# Autodesk Inventor assembly: Manipulator
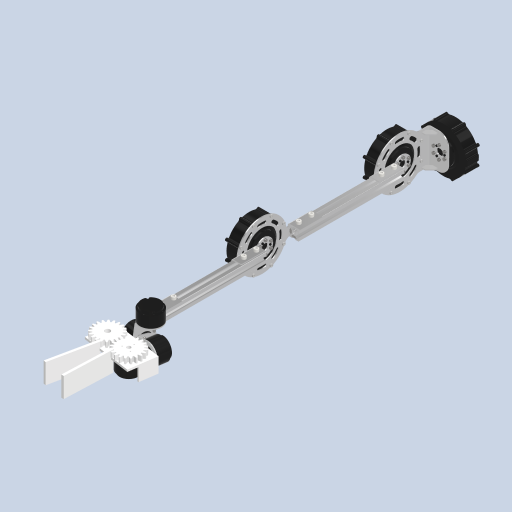
[picture p0: Inventor's stored thumbnail of the model, 512x512]
Saved by Autodesk Inventor 2023 (Build 270158000, 158)
## iProperties
Created: 2024-11-08
Part Number: Manipulator
Document SubType Name: Assembly
Designer: kiyo
Author: kiyo
## Documents named in this file (19)
- D:\GitHub\inventor\syu-si\OfficeRobot\Manipulator\Manipulator.iam
- D:\GitHub\inventor\syu-si\OfficeRobot\ReadyMade\Steadywin\GIM8108-8.iam
- D:\GitHub\inventor\syu-si\OfficeRobot\Manipulator\elbow-pitch-bracket.ipt
- D:\GitHub\inventor\syu-si\OfficeRobot\Manipulator\Hand.iam
- D:\GitHub\inventor\syu-si\OfficeRobot\ReadyMade\Screw\M3_6mm.ipt
- D:\GitHub\inventor\syu-si\OfficeRobot\ReadyMade\Steadywin\GIM3505-8_with-driver.ipt
- D:\GitHub\inventor\syu-si\OfficeRobot\Manipulator\wrist_roll_plate.ipt
- D:\GitHub\inventor\syu-si\OfficeRobot\Manipulator\wrist-pitch-plate.ipt
- D:\GitHub\inventor\syu-si\OfficeRobot\Manipulator\wrist-yaw-plate.ipt
- D:\GitHub\inventor\syu-si\OfficeRobot\ReadyMade\Screw\M2-5_6mm.ipt
- D:\GitHub\inventor\syu-si\OfficeRobot\ReadyMade\Screw\CBSH3-8.ipt
- D:\GitHub\inventor\syu-si\OfficeRobot\ReadyMade\Screw\FWSJJ-D5-V2_6-T4_5.ipt
- D:\GitHub\inventor\syu-si\OfficeRobot\ReadyMade\Screw\M2-5_10mm.ipt
- D:\GitHub\inventor\syu-si\OfficeRobot\ReadyMade\Screw\HNTU5-5.ipt
- D:\GitHub\inventor\syu-si\OfficeRobot\Manipulator\pitch_plate_20mm.ipt
- D:\GitHub\inventor\syu-si\OfficeRobot\ReadyMade\Aluminum-frame\HFS5-2020-210-AV10-BV35-CV175-DV200.ipt
- D:\GitHub\inventor\syu-si\OfficeRobot\Manipulator\sholder_roll_bracket.ipt
- D:\GitHub\inventor\syu-si\OfficeRobot\ReadyMade\Screw\SCB5-22.ipt
- D:\GitHub\inventor\syu-si\OfficeRobot\ReadyMade\Screw\SCB5-8.ipt
## Components (110 placed, 18 different names)
1. wrist_roll_plate:1 — 挿入:220, 挿入:227, 挿入:228, 挿入:229, 挿入:230, 挿入:231, 挿入:283, 挿入:284, 挿入:285
2. wrist-pitch-plate:1 — 挿入:211, 挿入:212, 挿入:213, 挿入:217, 挿入:218, 挿入:219, 挿入:220, 挿入:280, 挿入:281, 挿入:282
3. wrist-yaw-plate:1 — 挿入:203, 挿入:204, 挿入:205, 挿入:206, 挿入:207, 挿入:211, メイト:13, メイト:14, フラッシュ:4
4. pitch_plate_20mm:1 — 肩ピッチ, フラッシュ:1, 挿入:355, 挿入:356, 挿入:357, 挿入:358, 挿入:359, 挿入:360
5. pitch_plate_20mm:2 — 挿入:345, 肘ピッチ, フラッシュ:3
6. elbow-pitch-bracket:1 — 挿入:341, 挿入:342, フラッシュ:2, フラッシュ:7, フラッシュ:8
7. sholder_roll_bracket:1 — 挿入:348, 挿入:349, 挿入:350, 挿入:361, 挿入:362, 挿入:363, 挿入:364, 挿入:365, 挿入:366
8. Hand:1 [sub-assembly] — ハンド, 挿入:301
9. HFS5-2020-210-AV10-BV35-CV175-DV200:1 — フラッシュ:1, フラッシュ:2, メイト:19, メイト:20, 角度:35, 角度:36, メイト:21, メイト:22, フラッシュ:9, 角度:37, メイト:23, メイト:24
10. HFS5-2020-210-AV10-BV35-CV175-DV200:2 — フラッシュ:3, 挿入:351, 挿入:352, 角度:27, 角度:28, 挿入:353, 挿入:354, 角度:29, 角度:30, メイト:9, 角度:31, メイト:10, 角度:32, メイト:11, メイト:12, メイト:13, メイト:14, フラッシュ:4, メイト:15, メイト:16, 角度:33, フラッシュ:5, メイト:17, メイト:18, 角度:34, フラッシュ:6
11. M3_6mm:7 — 挿入:337
12. M3_6mm:8 — 挿入:336
13. M3_6mm:9 — 挿入:334
14. M3_6mm:10 — 挿入:338
15. M3_6mm:11 — 挿入:339
16. M3_6mm:12 — 挿入:335
17. M3_6mm:13
18. M3_6mm:14
19. M3_6mm:15
20. M3_6mm:16
21. M3_6mm:17
22. M3_6mm:18
23. M3_6mm:19 — 挿入:358
24. M3_6mm:20 — 挿入:357
25. M3_6mm:21 — 挿入:355
26. M3_6mm:22 — 挿入:356
27. M3_6mm:23 — 挿入:359
28. M3_6mm:24 — 挿入:360
29. M3_6mm:25 — 挿入:361
30. M3_6mm:26 — 挿入:363
31. M3_6mm:27 — 挿入:362
32. M3_6mm:28 — 挿入:364
33. M3_6mm:29 — 挿入:365
34. M3_6mm:30 — 挿入:366
35. CBSH3-8:1 — 挿入:307
36. CBSH3-8:2 — 挿入:308
37. CBSH3-8:3 — 挿入:302
38. CBSH3-8:4 — 挿入:304
39. CBSH3-8:5 — 挿入:309
40. CBSH3-8:6 — 挿入:303
41. CBSH3-8:7 — 挿入:305
42. CBSH3-8:8 — 挿入:306
43. CBSH3-8:9 — 挿入:332
44. CBSH3-8:10 — 挿入:327
45. CBSH3-8:11 — 挿入:330
46. CBSH3-8:12 — 挿入:328
47. CBSH3-8:13 — 挿入:329
48. CBSH3-8:14 — 挿入:331
49. CBSH3-8:15 — 挿入:326
50. CBSH3-8:16 — 挿入:333
51. M2-5_6mm:1 — 挿入:205
52. M2-5_6mm:2 — 挿入:207
53. M2-5_6mm:3 — 挿入:206
54. M2-5_6mm:7 — 挿入:229
55. M2-5_6mm:8 — 挿入:230
56. M2-5_6mm:9 — 挿入:231
57. M2-5_6mm:4 — 挿入:217
58. M2-5_6mm:5 — 挿入:218
59. M2-5_6mm:6 — 挿入:219
60. M2-5_10mm:1
61. M2-5_10mm:2
62. M2-5_10mm:3
63. M2-5_10mm:4
64. M2-5_10mm:5
65. M2-5_10mm:6
66. FWSJJ-D5-V2_6-T4_5:7 — 挿入:286
67. FWSJJ-D5-V2_6-T4_5:8 — 挿入:287
68. FWSJJ-D5-V2_6-T4_5:9 — 挿入:288
69. FWSJJ-D5-V2_6-T4_5:1 — 挿入:280
70. FWSJJ-D5-V2_6-T4_5:2 — 挿入:282
71. FWSJJ-D5-V2_6-T4_5:3 — 挿入:281
72. FWSJJ-D5-V2_6-T4_5:4 — 挿入:283
73. FWSJJ-D5-V2_6-T4_5:5 — 挿入:285
74. FWSJJ-D5-V2_6-T4_5:6 — 挿入:284
75. SCB5-22:1 — 挿入:368
76. SCB5-22:2 — 挿入:367
77. SCB5-22:3 — 挿入:370
78. SCB5-22:4 — 挿入:369
79. SCB5-22:5 — 挿入:372
80. SCB5-22:6 — 挿入:371
81. SCB5-22:7 — 挿入:376
82. SCB5-22:8 — 挿入:375
83. SCB5-8:1 — 挿入:374
84. SCB5-8:2 — 挿入:373
85. SCB5-8:3
86. SCB5-8:4
87. SCB5-8:5
88. SCB5-8:6
89. SCB5-8:7
90. HNTU5-5:6 — 挿入:372
91. HNTU5-5:7 — 挿入:371
92. HNTU5-5:9 — 挿入:369
93. HNTU5-5:10 — 挿入:370
94. HNTU5-5:11 — 挿入:351, 角度:28, 挿入:367
95. HNTU5-5:12 — 挿入:352, 角度:27, 挿入:368
96. HNTU5-5:13 — 挿入:353, 角度:30, 挿入:376
97. HNTU5-5:14 — 挿入:354, 角度:29, 挿入:375
98. HNTU5-5:15 — メイト:9, 角度:31, メイト:10, 挿入:373
99. HNTU5-5:16 — 角度:32, メイト:11, メイト:12, 挿入:374
100. HNTU5-5:17 — メイト:15, メイト:16, 角度:33, フラッシュ:5
101. HNTU5-5:18 — メイト:17, メイト:18, 角度:34, フラッシュ:6
102. HNTU5-5:19 — フラッシュ:8, メイト:19, メイト:20, 角度:35
103. HNTU5-5:20 — フラッシュ:7, 角度:36, メイト:21, メイト:22
104. HNTU5-5:21 — フラッシュ:9, 角度:37, メイト:23, メイト:24
105. GIM3505-8_with-driver:1 — 挿入:203, 挿入:204
106. GIM3505-8_with-driver:3 — 挿入:227, 挿入:228, 挿入:286, 挿入:287, 挿入:288, 挿入:301
107. GIM3505-8_with-driver:4 — 挿入:212, 挿入:213
108. GIM8108-8:1 [sub-assembly] — 挿入:350
109. GIM8108-8:2 [sub-assembly] — 挿入:302, 挿入:303, 挿入:304, 挿入:305, 挿入:306, 挿入:307, 挿入:308, 挿入:309, 挿入:348, 挿入:349
110. GIM8108-8:3 [sub-assembly] — 挿入:326, 挿入:327, 挿入:328, 挿入:329, 挿入:330, 挿入:331, 挿入:332, 挿入:333, 挿入:334, 挿入:335, 挿入:336, 挿入:337, 挿入:338, 挿入:339, 挿入:341, 挿入:342, 挿入:345
## Relationships (147: Insert 97, Mate 22, Angle 19, Flush 9)
- ハンド [Angle] (0 deg): Hand:1
- 挿入:203 [Insert]: wrist-yaw-plate:1 ↔ GIM3505-8_with-driver:1
- 挿入:204 [Insert]: wrist-yaw-plate:1 ↔ GIM3505-8_with-driver:1
- 挿入:205 [Insert]: wrist-yaw-plate:1 ↔ M2-5_6mm:1
- 挿入:206 [Insert]: wrist-yaw-plate:1 ↔ M2-5_6mm:3
- 挿入:207 [Insert]: wrist-yaw-plate:1 ↔ M2-5_6mm:2
- 挿入:211 [Insert] (3.5 mm): wrist-pitch-plate:1 ↔ wrist-yaw-plate:1
- 挿入:212 [Insert]: wrist-pitch-plate:1 ↔ GIM3505-8_with-driver:4
- 挿入:213 [Insert]: wrist-pitch-plate:1 ↔ GIM3505-8_with-driver:4
- 挿入:217 [Insert]: wrist-pitch-plate:1 ↔ M2-5_6mm:4
- 挿入:218 [Insert]: wrist-pitch-plate:1 ↔ M2-5_6mm:5
- 挿入:219 [Insert]: wrist-pitch-plate:1 ↔ M2-5_6mm:6
- 挿入:220 [Insert] (3.5 mm): wrist_roll_plate:1 ↔ wrist-pitch-plate:1
- [Insert]: wrist-pitch-plate:1 ↔ M2-5_10mm:1
- [Insert]: wrist-pitch-plate:1 ↔ M2-5_10mm:2
- [Insert]: wrist-pitch-plate:1 ↔ M2-5_10mm:3
- [Insert]: wrist_roll_plate:1 ↔ M2-5_10mm:6
- [Insert]: wrist_roll_plate:1 ↔ M2-5_10mm:4
- [Insert]: wrist_roll_plate:1 ↔ M2-5_10mm:5
- 挿入:227 [Insert]: wrist_roll_plate:1 ↔ GIM3505-8_with-driver:3
- 挿入:228 [Insert]: wrist_roll_plate:1 ↔ GIM3505-8_with-driver:3
- 挿入:229 [Insert]: wrist_roll_plate:1 ↔ M2-5_6mm:7
- 挿入:230 [Insert]: wrist_roll_plate:1 ↔ M2-5_6mm:8
- 挿入:231 [Insert]: wrist_roll_plate:1 ↔ M2-5_6mm:9
- 挿入:280 [Insert]: wrist-pitch-plate:1 ↔ FWSJJ-D5-V2_6-T4_5:1
- 挿入:281 [Insert]: wrist-pitch-plate:1 ↔ FWSJJ-D5-V2_6-T4_5:3
- 挿入:282 [Insert]: wrist-pitch-plate:1 ↔ FWSJJ-D5-V2_6-T4_5:2
- 挿入:283 [Insert]: wrist_roll_plate:1 ↔ FWSJJ-D5-V2_6-T4_5:4
- 挿入:284 [Insert]: wrist_roll_plate:1 ↔ FWSJJ-D5-V2_6-T4_5:6
- 挿入:285 [Insert]: wrist_roll_plate:1 ↔ FWSJJ-D5-V2_6-T4_5:5
- 挿入:286 [Insert]: FWSJJ-D5-V2_6-T4_5:7 ↔ GIM3505-8_with-driver:3
- 挿入:287 [Insert]: FWSJJ-D5-V2_6-T4_5:8 ↔ GIM3505-8_with-driver:3
- 挿入:288 [Insert]: FWSJJ-D5-V2_6-T4_5:9 ↔ GIM3505-8_with-driver:3
- 挿入:301 [Insert] (4.5 mm): Hand:1 ↔ GIM3505-8_with-driver:3
- 挿入:302 [Insert] (2 mm): CBSH3-8:3 ↔ GIM8108-8:2
- 挿入:303 [Insert] (2 mm): CBSH3-8:6 ↔ GIM8108-8:2
- 挿入:304 [Insert] (2 mm): CBSH3-8:4 ↔ GIM8108-8:2
- 挿入:305 [Insert] (2 mm): CBSH3-8:7 ↔ GIM8108-8:2
- 挿入:306 [Insert] (2 mm): CBSH3-8:8 ↔ GIM8108-8:2
- 挿入:307 [Insert] (2 mm): CBSH3-8:1 ↔ GIM8108-8:2
- 挿入:308 [Insert] (2 mm): CBSH3-8:2 ↔ GIM8108-8:2
- 挿入:309 [Insert] (2 mm): CBSH3-8:5 ↔ GIM8108-8:2
- [Insert] (-0.75 mm): HFS5-2020-210-AV10-BV35-CV175-DV200:1 ↔ HNTU5-5:6
- [Angle] (0 deg): HFS5-2020-210-AV10-BV35-CV175-DV200:1 ↔ HNTU5-5:6
- [Insert] (-0.75 mm): HFS5-2020-210-AV10-BV35-CV175-DV200:1 ↔ HNTU5-5:7
- [Angle] (0 deg): HFS5-2020-210-AV10-BV35-CV175-DV200:1 ↔ HNTU5-5:7
- [Angle] (0 deg): HFS5-2020-210-AV10-BV35-CV175-DV200:1 ↔ HNTU5-5:6
- 挿入:326 [Insert] (2 mm): CBSH3-8:15 ↔ GIM8108-8:3
- 挿入:327 [Insert] (2 mm): CBSH3-8:10 ↔ GIM8108-8:3
- 挿入:328 [Insert] (2 mm): CBSH3-8:12 ↔ GIM8108-8:3
- 挿入:329 [Insert] (2 mm): CBSH3-8:13 ↔ GIM8108-8:3
- 挿入:330 [Insert] (2 mm): CBSH3-8:11 ↔ GIM8108-8:3
- 挿入:331 [Insert] (2 mm): CBSH3-8:14 ↔ GIM8108-8:3
- 挿入:332 [Insert] (2 mm): CBSH3-8:9 ↔ GIM8108-8:3
- 挿入:333 [Insert] (2 mm): CBSH3-8:16 ↔ GIM8108-8:3
- 挿入:334 [Insert] (2 mm): M3_6mm:9 ↔ GIM8108-8:3
- 挿入:335 [Insert] (2 mm): M3_6mm:12 ↔ GIM8108-8:3
- 挿入:336 [Insert] (2 mm): M3_6mm:8 ↔ GIM8108-8:3
- 挿入:337 [Insert] (2 mm): M3_6mm:7 ↔ GIM8108-8:3
- 挿入:338 [Insert] (2 mm): M3_6mm:10 ↔ GIM8108-8:3
- 挿入:339 [Insert] (2 mm): M3_6mm:11 ↔ GIM8108-8:3
- [Insert]: pitch_plate_20mm:1 ↔ GIM8108-8:2
- [Mate]: pitch_plate_20mm:1 ↔ HFS5-2020-210-AV10-BV35-CV175-DV200:1
- [Mate]: pitch_plate_20mm:1 ↔ HFS5-2020-210-AV10-BV35-CV175-DV200:1
- 挿入:341 [Insert]: elbow-pitch-bracket:1 ↔ GIM8108-8:3
- 挿入:342 [Insert]: elbow-pitch-bracket:1 ↔ GIM8108-8:3
- [Angle] (0 deg): HFS5-2020-210-AV10-BV35-CV175-DV200:1 ↔ HNTU5-5:9
- [Angle] (0 deg): HFS5-2020-210-AV10-BV35-CV175-DV200:1 ↔ HNTU5-5:10
- [Insert] (-0.75 mm): HFS5-2020-210-AV10-BV35-CV175-DV200:1 ↔ HNTU5-5:9
- [Insert] (-0.75 mm): HFS5-2020-210-AV10-BV35-CV175-DV200:1 ↔ HNTU5-5:10
- [Mate]: elbow-pitch-bracket:1 ↔ HFS5-2020-210-AV10-BV35-CV175-DV200:1
- [Mate]: elbow-pitch-bracket:1 ↔ HFS5-2020-210-AV10-BV35-CV175-DV200:1
- 肩ピッチ [Angle] (0 deg): pitch_plate_20mm:1
- 挿入:345 [Insert]: pitch_plate_20mm:2 ↔ GIM8108-8:3
- [Mate]: pitch_plate_20mm:2 ↔ HFS5-2020-210-AV10-BV35-CV175-DV200:2
- [Mate]: pitch_plate_20mm:2 ↔ HFS5-2020-210-AV10-BV35-CV175-DV200:2
- 肘ピッチ [Angle] (0 deg): pitch_plate_20mm:2
- 挿入:348 [Insert]: sholder_roll_bracket:1 ↔ GIM8108-8:2
- 挿入:349 [Insert]: sholder_roll_bracket:1 ↔ GIM8108-8:2
- 挿入:350 [Insert]: sholder_roll_bracket:1 ↔ GIM8108-8:1
- フラッシュ:1 [Flush]: pitch_plate_20mm:1 ↔ HFS5-2020-210-AV10-BV35-CV175-DV200:1
- フラッシュ:2 [Flush]: elbow-pitch-bracket:1 ↔ HFS5-2020-210-AV10-BV35-CV175-DV200:1
- フラッシュ:3 [Flush]: pitch_plate_20mm:2 ↔ HFS5-2020-210-AV10-BV35-CV175-DV200:2
- 挿入:351 [Insert] (-0.75 mm): HFS5-2020-210-AV10-BV35-CV175-DV200:2 ↔ HNTU5-5:11
- 挿入:352 [Insert] (-0.75 mm): HFS5-2020-210-AV10-BV35-CV175-DV200:2 ↔ HNTU5-5:12
- 角度:27 [Angle] (0 deg): HFS5-2020-210-AV10-BV35-CV175-DV200:2 ↔ HNTU5-5:12
- 角度:28 [Angle] (0 deg): HFS5-2020-210-AV10-BV35-CV175-DV200:2 ↔ HNTU5-5:11
- 挿入:353 [Insert] (-0.75 mm): HFS5-2020-210-AV10-BV35-CV175-DV200:2 ↔ HNTU5-5:13
- 挿入:354 [Insert] (-0.75 mm): HFS5-2020-210-AV10-BV35-CV175-DV200:2 ↔ HNTU5-5:14
- 角度:29 [Angle] (0 deg): HFS5-2020-210-AV10-BV35-CV175-DV200:2 ↔ HNTU5-5:14
- 角度:30 [Angle] (0 deg): HFS5-2020-210-AV10-BV35-CV175-DV200:2 ↔ HNTU5-5:13
- メイト:9 [Mate]: HFS5-2020-210-AV10-BV35-CV175-DV200:2 ↔ HNTU5-5:15
- 角度:31 [Angle] (0 deg): HFS5-2020-210-AV10-BV35-CV175-DV200:2 ↔ HNTU5-5:15
- メイト:10 [Mate] (0.1 mm): HFS5-2020-210-AV10-BV35-CV175-DV200:2 ↔ HNTU5-5:15
- 角度:32 [Angle] (0 deg): HFS5-2020-210-AV10-BV35-CV175-DV200:2 ↔ HNTU5-5:16
- メイト:11 [Mate]: HFS5-2020-210-AV10-BV35-CV175-DV200:2 ↔ HNTU5-5:16
- メイト:12 [Mate] (0.1 mm): HFS5-2020-210-AV10-BV35-CV175-DV200:2 ↔ HNTU5-5:16
- 挿入:355 [Insert]: pitch_plate_20mm:1 ↔ M3_6mm:21
- 挿入:356 [Insert]: pitch_plate_20mm:1 ↔ M3_6mm:22
- 挿入:357 [Insert]: pitch_plate_20mm:1 ↔ M3_6mm:20
- 挿入:358 [Insert]: pitch_plate_20mm:1 ↔ M3_6mm:19
- 挿入:359 [Insert]: pitch_plate_20mm:1 ↔ M3_6mm:23
- 挿入:360 [Insert]: pitch_plate_20mm:1 ↔ M3_6mm:24
- 挿入:361 [Insert]: sholder_roll_bracket:1 ↔ M3_6mm:25
- 挿入:362 [Insert]: sholder_roll_bracket:1 ↔ M3_6mm:27
- 挿入:363 [Insert]: sholder_roll_bracket:1 ↔ M3_6mm:26
- 挿入:364 [Insert]: sholder_roll_bracket:1 ↔ M3_6mm:28
- 挿入:365 [Insert]: sholder_roll_bracket:1 ↔ M3_6mm:29
- 挿入:366 [Insert]: sholder_roll_bracket:1 ↔ M3_6mm:30
- 挿入:367 [Insert] (-1.25 mm): SCB5-22:2 ↔ HNTU5-5:11
- 挿入:368 [Insert] (-1.25 mm): SCB5-22:1 ↔ HNTU5-5:12
- 挿入:369 [Insert] (-1.25 mm): SCB5-22:4 ↔ HNTU5-5:9
- 挿入:370 [Insert] (-1.25 mm): SCB5-22:3 ↔ HNTU5-5:10
- 挿入:371 [Insert] (-1.25 mm): SCB5-22:6 ↔ HNTU5-5:7
- 挿入:372 [Insert] (-1.25 mm): SCB5-22:5 ↔ HNTU5-5:6
- 挿入:373 [Insert] (3.2 mm): SCB5-8:2 ↔ HNTU5-5:15
- 挿入:374 [Insert] (3.2 mm): SCB5-8:1 ↔ HNTU5-5:16
- メイト:13 [Mate]: wrist-yaw-plate:1 ↔ HFS5-2020-210-AV10-BV35-CV175-DV200:2
- メイト:14 [Mate]: wrist-yaw-plate:1 ↔ HFS5-2020-210-AV10-BV35-CV175-DV200:2
- フラッシュ:4 [Flush]: wrist-yaw-plate:1 ↔ HFS5-2020-210-AV10-BV35-CV175-DV200:2
- 挿入:375 [Insert] (-1.25 mm): SCB5-22:8 ↔ HNTU5-5:14
- 挿入:376 [Insert] (-1.25 mm): SCB5-22:7 ↔ HNTU5-5:13
- [Insert] (3.2 mm): SCB5-8:3 ↔ HNTU5-5:17
- メイト:15 [Mate]: HFS5-2020-210-AV10-BV35-CV175-DV200:2 ↔ HNTU5-5:17
- メイト:16 [Mate] (1 mm): HFS5-2020-210-AV10-BV35-CV175-DV200:2 ↔ HNTU5-5:17
- 角度:33 [Angle] (0 deg): HFS5-2020-210-AV10-BV35-CV175-DV200:2 ↔ HNTU5-5:17
- フラッシュ:5 [Flush] (33.5 mm): HFS5-2020-210-AV10-BV35-CV175-DV200:2 ↔ HNTU5-5:17
- [Insert] (3.2 mm): SCB5-8:4 ↔ HNTU5-5:18
- メイト:17 [Mate]: HFS5-2020-210-AV10-BV35-CV175-DV200:2 ↔ HNTU5-5:18
- メイト:18 [Mate] (1 mm): HFS5-2020-210-AV10-BV35-CV175-DV200:2 ↔ HNTU5-5:18
- 角度:34 [Angle] (0 deg): HFS5-2020-210-AV10-BV35-CV175-DV200:2 ↔ HNTU5-5:18
- フラッシュ:6 [Flush] (33.5 mm): HFS5-2020-210-AV10-BV35-CV175-DV200:2 ↔ HNTU5-5:18
- [Insert] (3.2 mm): SCB5-8:5 ↔ HNTU5-5:19
- [Insert] (3.2 mm): SCB5-8:6 ↔ HNTU5-5:20
- フラッシュ:7 [Flush] (5.5 mm): elbow-pitch-bracket:1 ↔ HNTU5-5:20
- フラッシュ:8 [Flush] (-30.5 mm): elbow-pitch-bracket:1 ↔ HNTU5-5:19
- メイト:19 [Mate]: HFS5-2020-210-AV10-BV35-CV175-DV200:1 ↔ HNTU5-5:19
- メイト:20 [Mate] (1 mm): HFS5-2020-210-AV10-BV35-CV175-DV200:1 ↔ HNTU5-5:19
- 角度:35 [Angle] (0 deg): HFS5-2020-210-AV10-BV35-CV175-DV200:1 ↔ HNTU5-5:19
- 角度:36 [Angle] (0 deg): HFS5-2020-210-AV10-BV35-CV175-DV200:1 ↔ HNTU5-5:20
- メイト:21 [Mate] (1 mm): HFS5-2020-210-AV10-BV35-CV175-DV200:1 ↔ HNTU5-5:20
- メイト:22 [Mate]: HFS5-2020-210-AV10-BV35-CV175-DV200:1 ↔ HNTU5-5:20
- [Insert] (3.2 mm): SCB5-8:7 ↔ HNTU5-5:21
- フラッシュ:9 [Flush] (33.5 mm): HFS5-2020-210-AV10-BV35-CV175-DV200:1 ↔ HNTU5-5:21
- 角度:37 [Angle] (0 deg): HFS5-2020-210-AV10-BV35-CV175-DV200:1 ↔ HNTU5-5:21
- メイト:23 [Mate] (1 mm): HFS5-2020-210-AV10-BV35-CV175-DV200:1 ↔ HNTU5-5:21
- メイト:24 [Mate]: HFS5-2020-210-AV10-BV35-CV175-DV200:1 ↔ HNTU5-5:21
## Named parameters: d472_d466 = 3.2 mm, d477_d466 = 3.2 mm, d482_d466 = 3.2 mm, d483_d466 = 3.2 mm, d492_d466 = 3.2 mm
